# Autodesk Inventor assembly: Printhead Assembly Autolevel
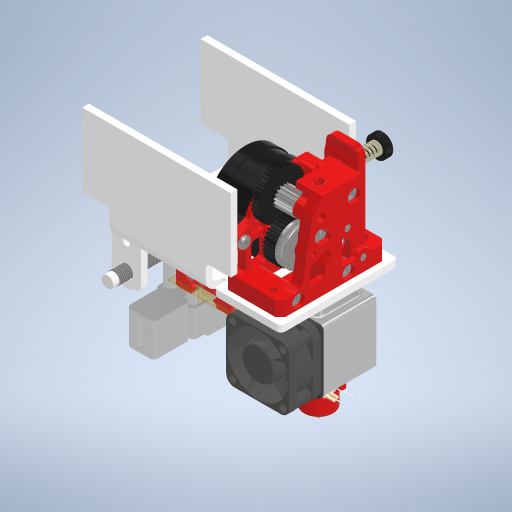
[picture p0: Inventor's stored thumbnail of the model, 512x512]
Saved by Autodesk Inventor 2024 (Build 280153000, 153)
## iProperties
Created: 2024-12-30
Part Number: Printhead Assembly Autolevel
Document SubType Name: Assembly
Designer: Ishaan
Author: Ishaan
## Documents named in this file (16)
- E:\Projects\Axiom--IDEX-3D-Printer\CAD\05 - Printhead\Printhead Assembly Autolevel.iam
- E:\Projects\Axiom--IDEX-3D-Printer\CAD\00 - COTS Components\MGN12H\MGN12H, LINEAR GUIDE BLOCK.ipt
- E:\Projects\Axiom--IDEX-3D-Printer\CAD\05 - Printhead\Printhead Baseplate.ipt
- E:\Projects\Axiom--IDEX-3D-Printer\CAD\00 - COTS Components\HGXLite Extruder\HGX-extruder\HGX-extruder.ipt
- E:\Projects\Axiom--IDEX-3D-Printer\CAD\00 - COTS Components\6mm Inductive Probe\6mm Inductive Probe.ipt
- E:\Projects\Axiom--IDEX-3D-Printer\CAD\00 - COTS Components\CHC Hotend\TD6S-CHC_mockup.iam
- E:\Projects\Axiom--IDEX-3D-Printer\CAD\05 - Printhead\Printhead Belt Retainer Cap.ipt
- E:\Projects\Axiom--IDEX-3D-Printer\CAD\05 - Printhead\Printhead Belt Retainer R2.ipt
- E:\Projects\Axiom--IDEX-3D-Printer\CAD\00 - COTS Components\3015 Fan\3015 Fan.ipt
- E:\Projects\Axiom--IDEX-3D-Printer\CAD\00 - COTS Components\Hardware\M3 25mm Standoff.ipt
- E:\Projects\Axiom--IDEX-3D-Printer\CAD\00 - COTS Components\Hardware\M3 10mm Standoff.ipt
- E:\Projects\Axiom--IDEX-3D-Printer\CAD\05 - Printhead\Inductive Probe Mount.ipt
- E:\Projects\Axiom--IDEX-3D-Printer\CAD\05 - Printhead\Hotend Cooling Fan Mount.ipt
- E:\Projects\Axiom--IDEX-3D-Printer\CAD\05 - Printhead\Hotend Cooling Fan Gasket.ipt
- E:\Projects\Axiom--IDEX-3D-Printer\CAD\00 - COTS Components\5015 Fan\Radial-Cooling-Fan-5015-DC12V.iam
- E:\Projects\Axiom--IDEX-3D-Printer\CAD\05 - Printhead\Printhead Cover Duct.ipt
## Components (28 placed, 15 different names)
1. MGN12H, LINEAR GUIDE BLOCK:1 — Insert:23, Insert:24
2. Printhead Baseplate:1 — Insert:9, Insert:10, Insert:23, Insert:24, Insert:65, Insert:66, Insert:67, Insert:68, Insert:70, Insert:71, Angle:2
3. HGX-extruder:1 — Insert:9, Insert:10
4. 6mm Inductive Probe:1 — Mate:1, Flush:1
5. TD6S-CHC_mockup:1 [sub-assembly] — Insert:72, Insert:73, Mate:4, Mate:6
6. 3015 Fan:1 — Insert:76, Insert:77
7. Inductive Probe Mount:1 — Insert:67, Insert:68, Mate:1, Flush:1, Insert:69
8. M3 25mm Standoff:5 — Insert:69
9. Hotend Cooling Fan Mount:1 — Insert:70, Insert:71, Insert:72, Insert:73, Insert:74, Insert:75, Mate:7
10. Hotend Cooling Fan Gasket:1 — Insert:74, Insert:75, Insert:76, Insert:77
11. Radial-Cooling-Fan-5015-DC12V:1 [sub-assembly] — Mate:8, Mate:9
12. Printhead Cover Duct:1 — Mate:6, Mate:7, Mate:8, Mate:9
13. Printhead Belt Retainer Cap:5
14. Printhead Belt Retainer R2:5 — Insert:61, Insert:62, Insert:63, Insert:64
15. Printhead Belt Retainer Cap:6
16. Printhead Belt Retainer R2:6
17. M3 10mm Standoff:1 — Insert:64, Insert:65
18. M3 10mm Standoff:2 — Insert:63
19. M3 10mm Standoff:3 — Insert:62
20. M3 10mm Standoff:4 — Insert:61, Insert:66
21. M3 25mm Standoff:1
22. M3 25mm Standoff:2 — Insert:51
23. M3 25mm Standoff:3
24. M3 25mm Standoff:4 — Insert:52
25. Printhead Belt Retainer Cap:3 — Insert:45, Insert:46
26. Printhead Belt Retainer R2:3 — Insert:45, Insert:46, Insert:51, Insert:52
27. Printhead Belt Retainer Cap:4 — Insert:49, Insert:50
28. Printhead Belt Retainer R2:4 — Insert:49, Insert:50
## Relationships (49: Insert 39, Mate 7, Flush 2, Angle 1)
- Insert:9: Printhead Baseplate:1 ↔ HGX-extruder:1
- Insert:10: Printhead Baseplate:1 ↔ HGX-extruder:1
- Insert:23: MGN12H, LINEAR GUIDE BLOCK:1 ↔ Printhead Baseplate:1
- Insert:24: MGN12H, LINEAR GUIDE BLOCK:1 ↔ Printhead Baseplate:1
- [Insert]: Printhead Baseplate:1 ↔ M3 25mm Standoff:4
- [Insert]: Printhead Baseplate:1 ↔ M3 25mm Standoff:3
- [Insert]: Printhead Baseplate:1 ↔ M3 25mm Standoff:2
- [Insert]: Printhead Baseplate:1 ↔ M3 25mm Standoff:1
- Insert:45: Printhead Belt Retainer Cap:3 ↔ Printhead Belt Retainer R2:3
- Insert:46: Printhead Belt Retainer Cap:3 ↔ Printhead Belt Retainer R2:3
- [Insert]: Printhead Belt Retainer R2:3 ↔ Printhead Belt Retainer R2:4
- [Insert]: Printhead Belt Retainer R2:3 ↔ Printhead Belt Retainer R2:4
- Insert:49: Printhead Belt Retainer Cap:4 ↔ Printhead Belt Retainer R2:4
- Insert:50: Printhead Belt Retainer Cap:4 ↔ Printhead Belt Retainer R2:4
- Insert:51: M3 25mm Standoff:2 ↔ Printhead Belt Retainer R2:3
- Insert:52: M3 25mm Standoff:4 ↔ Printhead Belt Retainer R2:3
- [Insert]: Printhead Belt Retainer Cap:5 ↔ Printhead Belt Retainer R2:5
- [Insert]: Printhead Belt Retainer Cap:5 ↔ Printhead Belt Retainer R2:5
- [Insert]: Printhead Belt Retainer R2:5 ↔ Printhead Belt Retainer R2:6
- [Insert]: Printhead Belt Retainer R2:5 ↔ Printhead Belt Retainer R2:6
- [Insert]: Printhead Belt Retainer Cap:6 ↔ Printhead Belt Retainer R2:6
- [Insert]: Printhead Belt Retainer Cap:6 ↔ Printhead Belt Retainer R2:6
- Insert:61: Printhead Belt Retainer R2:5 ↔ M3 10mm Standoff:4
- Insert:62: Printhead Belt Retainer R2:5 ↔ M3 10mm Standoff:3
- Insert:63: Printhead Belt Retainer R2:5 ↔ M3 10mm Standoff:2
- Insert:64: Printhead Belt Retainer R2:5 ↔ M3 10mm Standoff:1
- Insert:65: Printhead Baseplate:1 ↔ M3 10mm Standoff:1
- Insert:66: Printhead Baseplate:1 ↔ M3 10mm Standoff:4
- Insert:67: Printhead Baseplate:1 ↔ Inductive Probe Mount:1
- Insert:68: Printhead Baseplate:1 ↔ Inductive Probe Mount:1
- Mate:1: 6mm Inductive Probe:1 ↔ Inductive Probe Mount:1
- Flush:1 (9 mm): 6mm Inductive Probe:1 ↔ Inductive Probe Mount:1
- Insert:69: Inductive Probe Mount:1 ↔ M3 25mm Standoff:5
- Insert:70: Printhead Baseplate:1 ↔ Hotend Cooling Fan Mount:1
- Insert:71: Printhead Baseplate:1 ↔ Hotend Cooling Fan Mount:1
- Insert:72: TD6S-CHC_mockup:1 ↔ Hotend Cooling Fan Mount:1
- Insert:73: TD6S-CHC_mockup:1 ↔ Hotend Cooling Fan Mount:1
- Insert:74: Hotend Cooling Fan Mount:1 ↔ Hotend Cooling Fan Gasket:1
- Insert:75: Hotend Cooling Fan Mount:1 ↔ Hotend Cooling Fan Gasket:1
- Insert:76: 3015 Fan:1 ↔ Hotend Cooling Fan Gasket:1
- Insert:77: 3015 Fan:1 ↔ Hotend Cooling Fan Gasket:1
- Mate:4: TD6S-CHC_mockup:1
- Mate:5
- Angle:2 (0 deg): Printhead Baseplate:1
- Flush:2 (-17 mm)
- Mate:6: TD6S-CHC_mockup:1 ↔ Printhead Cover Duct:1
- Mate:7: Hotend Cooling Fan Mount:1 ↔ Printhead Cover Duct:1
- Mate:8: Radial-Cooling-Fan-5015-DC12V:1 ↔ Printhead Cover Duct:1
- Mate:9: Radial-Cooling-Fan-5015-DC12V:1 ↔ Printhead Cover Duct:1
## Named parameters: d45_d31 = 0 mm, d46_d32 = 0 mm, d47_d33 = 0 mm, d48_d34 = 0 mm, d49_d35 = 0 mm, d50_d36 = 0 mm, d55_d45_d31 = 0 mm, d56_d46_d32 = 0 mm, d57_d47_d33 = 0 mm, d58_d48_d34 = 0 mm, d59_d49_d35 = 0 mm, d60_d50_d36 = 0 mm
